# Autodesk Inventor assembly: RoadBot Pneumatic Module - with Jack - r1
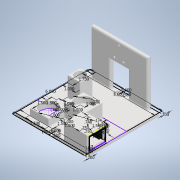
[picture p0: Inventor's stored thumbnail of the model, 180x180]
Saved by Autodesk Inventor 2020 (Build 240168000, 168)
## iProperties
Created: 2022-04-02
Part Number: RoadBot Pneumatic Module - with Jack - r1
Document SubType Name: Assembly
Designer: Beaucage
Author: Beaucage
## Documents named in this file (3)
- V:\AFL\Drawings\RoadBot Pneumatic Module - with Jack - r1.iam
- V:\AFL\Drawings\RoadBot Pneumatic Module - Base - r1.ipt
- V:\AFL\Drawings\Keystone_Jack_Single_Receptacle (1).ipt
## Components (2 placed, 2 different names)
1. RoadBot Pneumatic Module - Base - r1:1 — Mate:1, Mate:2, Flush:1
2. Keystone_Jack_Single_Receptacle (1):1 — Mate:1, Mate:2, Flush:1
## Relationships (3: Mate 2, Flush 1)
- Mate:1: RoadBot Pneumatic Module - Base - r1:1 ↔ Keystone_Jack_Single_Receptacle (1):1
- Mate:2: RoadBot Pneumatic Module - Base - r1:1 ↔ Keystone_Jack_Single_Receptacle (1):1
- Flush:1: RoadBot Pneumatic Module - Base - r1:1 ↔ Keystone_Jack_Single_Receptacle (1):1
